# Autodesk Inventor assembly: Wheel Assembly
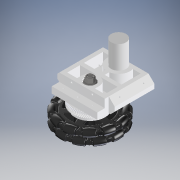
[picture p0: Inventor's stored thumbnail of the model, 180x180]
Saved by Autodesk Inventor 2017 SP1 (Build 210196100, 196)
## iProperties
Created: 2017-08-01
Part Number: Wheel Assembly
Document SubType Name: Assembly
Designer: Zach
Author: Zach
## Documents named in this file (12)
- C:\Users\Zach\Documents\GitHub\tr1\src\Base\Wheel Assembly\Wheel Assembly.iam
- C:\Users\Zach\Documents\GitHub\tr1\lib\Omni Wheel 6in\217-2585.ipt
- C:\Users\Zach\Documents\GitHub\tr1\lib\28x12x8mm Bearing.ipt
- C:\Users\Zach\Documents\GitHub\tr1\src\Base\Wheel Assembly\WA004.ipt
- C:\Users\Zach\Documents\GitHub\tr1\src\Base\Wheel Assembly\Wheel Assembly\Design Accelerator\Spur Gears1.iam
- C:\Users\Zach\Documents\GitHub\tr1\src\Base\Wheel Assembly\WA002.ipt
- C:\Users\Zach\Documents\GitHub\tr1\lib\AS 1110 - M12 x 100.ipt
- C:\Users\Zach\Documents\GitHub\tr1\lib\ISO 4032 - M12 - ISO.ipt
- C:\Users\Zach\Documents\GitHub\tr1\lib\6mm Mounting Hub.ipt
- C:\Users\Zach\Documents\GitHub\tr1\lib\12V DC Motor\12V DC Motor.iam
- C:\Users\Zach\Documents\GitHub\tr1\src\Base\Wheel Assembly\Small Gear.iam
- C:\Users\Zach\Documents\GitHub\tr1\src\Base\Wheel Assembly\Wheel Assembly\Design Accelerator\Spur Gears3.iam
## Components (14 placed, 10 different names)
1. 217-2585:1 — Mate:1, Flush:1, Mate:2, Flush:2, Mate:27, Mate:28, Mate:34, Mate:79
2. 28x12x8mm Bearing:1 — Mate:1, Flush:1, Mate:32
3. 28x12x8mm Bearing:2 — Mate:2, Flush:2, Mate:43, Mate:44, Mate:47
4. WA004:1 — Mate:17, Mate:18, Mate:19, Mate:20, Mate:34, Mate:35, Mate:42, Mate:56, Mate:57, Mate:62, Mate:67, Mate:68, Mate:69, Mate:70, Mate:71, Mate:72, Mate:74
5. 28x12x8mm Bearing:3 — Mate:19, Mate:20
6. 28x12x8mm Bearing:4 — Mate:17, Mate:18, Mate:46
7. Spur Gears:1 [sub-assembly] — Mate:27, Mate:28, Mate:35, Mate:61, Mate:62, Mate:63, Mate:71, Mate:72
8. WA002:1 — Mate:32, Mate:47
9. AS 1110 - Metric M12 x 100:1 — Mate:43, Mate:44, Mate:45, Mate:51, Mate:52, Mate:73
10. ISO 4032 M12:1 — Mate:45, Mate:46
11. 6mm Mounting Hub:1 — Mate:56, Mate:57, Mate:61, Mate:63, Mate:75, Mate:77, Mate:78
12. 12V DC Motor:1 [sub-assembly] — Mate:67, Mate:68, Mate:69, Mate:76
13. Small Gear:1 [sub-assembly] — Mate:73, Mate:74, Rotation:1, Mate:79
14. Spur Gears:2 [sub-assembly] — Mate:75, Mate:76, Mate:77, Mate:78, Rotation:1
## Relationships (40: Mate 37, Flush 2, RelateRotation 1)
- Mate:1: 217-2585:1 ↔ 28x12x8mm Bearing:1
- Flush:1: 217-2585:1 ↔ 28x12x8mm Bearing:1
- Mate:2: 217-2585:1 ↔ 28x12x8mm Bearing:2
- Flush:2: 217-2585:1 ↔ 28x12x8mm Bearing:2
- Mate:17: WA004:1 ↔ 28x12x8mm Bearing:4
- Mate:18: WA004:1 ↔ 28x12x8mm Bearing:4
- Mate:19: WA004:1 ↔ 28x12x8mm Bearing:3
- Mate:20: WA004:1 ↔ 28x12x8mm Bearing:3
- Mate:27: 217-2585:1 ↔ Spur Gears:1
- Mate:28: 217-2585:1 ↔ Spur Gears:1
- Mate:32: 28x12x8mm Bearing:1 ↔ WA002:1
- Mate:34: 217-2585:1 ↔ WA004:1
- Mate:35: WA004:1 ↔ Spur Gears:1
- Mate:42: WA004:1
- Mate:43: 28x12x8mm Bearing:2 ↔ AS 1110 - Metric M12 x 100:1
- Mate:44: 28x12x8mm Bearing:2 ↔ AS 1110 - Metric M12 x 100:1
- Mate:45: AS 1110 - Metric M12 x 100:1 ↔ ISO 4032 M12:1
- Mate:46: 28x12x8mm Bearing:4 ↔ ISO 4032 M12:1
- Mate:47: 28x12x8mm Bearing:2 ↔ WA002:1
- Mate:51: AS 1110 - Metric M12 x 100:1
- Mate:52: AS 1110 - Metric M12 x 100:1
- Mate:56: WA004:1 ↔ 6mm Mounting Hub:1
- Mate:57: WA004:1 ↔ 6mm Mounting Hub:1
- Mate:61: Spur Gears:1 ↔ 6mm Mounting Hub:1
- Mate:62: WA004:1 ↔ Spur Gears:1
- Mate:63: Spur Gears:1 ↔ 6mm Mounting Hub:1
- Mate:67: WA004:1 ↔ 12V DC Motor:1
- Mate:68: WA004:1 ↔ 12V DC Motor:1
- Mate:69: WA004:1 ↔ 12V DC Motor:1
- Mate:70: WA004:1
- Mate:71: WA004:1 ↔ Spur Gears:1
- Mate:72: WA004:1 ↔ Spur Gears:1
- Mate:73: AS 1110 - Metric M12 x 100:1 ↔ Small Gear:1
- Mate:74: WA004:1 ↔ Small Gear:1
- Mate:75: 6mm Mounting Hub:1 ↔ Spur Gears:2
- Mate:76: 12V DC Motor:1 ↔ Spur Gears:2
- Mate:77: 6mm Mounting Hub:1 ↔ Spur Gears:2
- Mate:78: 6mm Mounting Hub:1 ↔ Spur Gears:2
- Rotation:1 [RelateRotation] (0.506 ul): Small Gear:1 ↔ Spur Gears:2
- Mate:79: 217-2585:1 ↔ Small Gear:1
